# Autodesk Inventor assembly: Assembly15
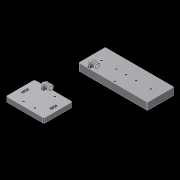
[picture p0: Inventor's stored thumbnail of the model, 180x180]
Saved by Autodesk Inventor 2021.1 (Build 251245010, 245A)
## iProperties
Created: 2020-11-02
Part Number: Assembly15
Document SubType Name: Assembly
Designer: Hashimoto
Author: Hashimoto
## Documents named in this file (4)
- Z:\inventorroom\sample\unit4\Assembly15.iam
- Z:\inventorroom\sample\unit4\01.ipt
- Z:\inventorroom\sample\unit4\02.ipt
- Z:\inventorroom\sample\unit4\KJL06-M5.ipt
## Components (4 placed, 3 different names)
1. 01:1 — 挿入:1
2. 02:1 — 挿入:2
3. KJL06-M5:1 — 挿入:1
4. KJL06-M5:2 — 挿入:2
## Relationships (2: Insert 2)
- 挿入:1 [Insert]: 01:1 ↔ KJL06-M5:1
- 挿入:2 [Insert]: 02:1 ↔ KJL06-M5:2
